# Autodesk Inventor assembly: Ensamble_general
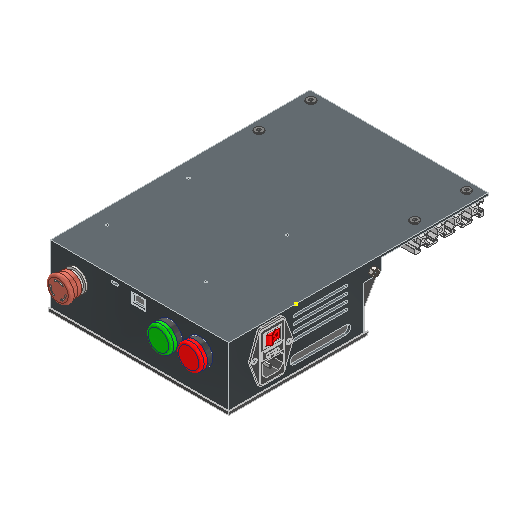
[picture p0: Inventor's stored thumbnail of the model, 512x512]
Saved by Autodesk Inventor 2025 (Build 290162000, 162)
## iProperties
Created: 2026-01-23
Part Number: Ensamble_general
Document SubType Name: Assembly
Designer: HP
Author: HP
## Documents named in this file (24)
- C:\Users\HP\Desktop\TESIS 2\TFC2_20212123_MHinojosa\TFC2-20212123-HW\CAD\Ensamble_general.iam
- C:\Users\HP\Desktop\TESIS 2\TFC2_20212123_MHinojosa\TFC2-20212123-HW\CAD\Chasis\Chasis_CONTROL.ipt
- C:\Users\HP\Desktop\TESIS 2\TFC2_20212123_MHinojosa\TFC2-20212123-HW\CAD\AC_INTERUP\AC_INTERUP.ipt
- C:\Users\HP\Desktop\TESIS 2\TFC2_20212123_MHinojosa\TFC2-20212123-HW\CAD\Banana Socket (Red)\Banana Socket (Red).ipt
- C:\Users\HP\Desktop\TESIS 2\TFC2_20212123_MHinojosa\TFC2-20212123-HW\CAD\Banana Socket (Black)\Banana Socket (Black).ipt
- C:\Users\HP\Desktop\TESIS 2\TFC2_20212123_MHinojosa\TFC2-20212123-HW\CAD\RED LED BULB_F\RED LED BULB_F.ipt
- C:\Users\HP\Desktop\TESIS 2\TFC2_20212123_MHinojosa\TFC2-20212123-HW\CAD\GREEN LED BULB_F\GREEN LED BULB_F.ipt
- C:\Users\HP\Desktop\TESIS 2\TFC2_20212123_MHinojosa\TFC2-20212123-HW\CAD\Profiles\Profiles.ipt
- C:\Users\HP\Desktop\TESIS 2\TFC2_20212123_MHinojosa\TFC2-20212123-HW\CAD\E-Stop\E-Stop.ipt
- C:\Users\HP\Desktop\TESIS 2\TFC2_20212123_MHinojosa\TFC2-20212123-HW\CAD\Tapa_chasis.ipt
- C:\Users\HP\Desktop\TESIS 2\TFC2_20212123_MHinojosa\TFC2-20212123-HW\CAD\BRACKET_MOTOR.ipt
- C:\Users\HP\Desktop\TESIS 2\TFC2_20212123_MHinojosa\TFC2-20212123-HW\CAD\DC Planetary Gear Brush Motor (PZ22GR9120R-084BBH)\DC Planetary Gear Brush Motor (PZ22GR9120R-084BBH).ipt
- C:\Users\HP\Desktop\TESIS 2\TFC2_20212123_MHinojosa\TFC2-20212123-HW\CAD\Slider T-Nut for 2020 - M5\Slider T-Nut for 2020 - M5.ipt
- C:\Users\HP\Desktop\TESIS 2\TFC2_20212123_MHinojosa\TFC2-20212123-HW\CAD\TORNILLO ALLEN CABEZA PLANA M3x0.5x6\TORNILLO ALLEN CABEZA PLANA M5x0.5x6.ipt
- C:\Users\HP\Desktop\TESIS 2\TFC2_20212123_MHinojosa\TFC2-20212123-HW\CAD\BRACKET_SENSOR.ipt
- C:\Users\HP\Desktop\TESIS 2\TFC2_20212123_MHinojosa\TFC2-20212123-HW\CAD\3D_PCB3_2026-01-02\3D_PCB3_2026-01-02.iam
- C:\Users\HP\Desktop\TESIS 2\TFC2_20212123_MHinojosa\TFC2-20212123-HW\CAD\Acople_IMAN_SOLO.ipt
- C:\Users\HP\Desktop\TESIS 2\TFC2_20212123_MHinojosa\TFC2-20212123-HW\CAD\M3x5\M3x5.ipt
- C:\Users\HP\Desktop\TESIS 2\TFC2_20212123_MHinojosa\TFC2-20212123-HW\CAD\M3 nut\M3 nut.ipt
- C:\Users\HP\Desktop\TESIS 2\TFC2_20212123_MHinojosa\TFC2-20212123-HW\CAD\M5x10\M5x10.ipt
- C:\Users\HP\Desktop\TESIS 2\TFC2_20212123_MHinojosa\TFC2-20212123-HW\CAD\M5 Nut\M5 Nut.ipt
- C:\Users\HP\Desktop\TESIS 2\TFC2_20212123_MHinojosa\TFC2-20212123-HW\CAD\M3 x 10 Brass Standoff_\M3 x 10 Brass Standoff_.ipt
- C:\Users\HP\Desktop\TESIS 2\TFC2_20212123_MHinojosa\TFC2-20212123-HW\CAD\3D_PCB10_2026-02-04\3D_PCB10_2026-02-04.ipt
- C:\Users\HP\Desktop\TESIS 2\TFC2_20212123_MHinojosa\TFC2-20212123-HW\CAD\FuenteConmutada24W\FuenteConmutada12V2A\FuenteConmutada12V2A.ipt
## Components (54 placed, 23 different names)
1. Chasis_CONTROL:1 — Coincidencia:1, Coincidencia:2, Coincidencia:3, Coincidencia:9, Coincidencia:10, Coincidencia:11, Coincidencia:12, Nivelación:1, Coincidencia:14, Nivelación:2, Coincidencia:19, Coincidencia:20, Coincidencia:21, Coincidencia:22, Coincidencia:23, Coincidencia:34, Coincidencia:37, Coincidencia:39, Coincidencia:41, Coincidencia:50, Coincidencia:51, Coincidencia:52, Coincidencia:53, Coincidencia:54, Coincidencia:55, Coincidencia:56, Coincidencia:57, Ángulo:1, Ángulo:2, Ángulo:3, Ángulo:4, Ángulo:5, Ángulo:6, Ángulo:7, Ángulo:8, Ángulo:9, Ángulo:10, Coincidencia:124, Coincidencia:127, Coincidencia:129, Coincidencia:134, Coincidencia:135, Ángulo:11, Ángulo:12, Coincidencia:136, Coincidencia:137, Coincidencia:138, Coincidencia:139, Ángulo:13, Ángulo:14, Ángulo:15, Coincidencia:140, Coincidencia:141, Coincidencia:142, Coincidencia:143, Coincidencia:144, Coincidencia:148, Coincidencia:149, Nivelación:13
2. AC_INTERUP:1 — Coincidencia:1, Coincidencia:2, Coincidencia:3
3. RED LED BULB_F:1 — Coincidencia:9, Coincidencia:12, Ángulo:15
4. GREEN LED BULB_F:1 — Coincidencia:10, Coincidencia:11, Ángulo:14
5. Profiles:1 — Nivelación:1, Coincidencia:14, Nivelación:2, Nivelación:5, Coincidencia:28, Nivelación:6, Coincidencia:32, Coincidencia:33, Coincidencia:36, Coincidencia:38, Coincidencia:40, Coincidencia:42, Coincidencia:44, Coincidencia:46, Coincidencia:48, Coincidencia:93, Nivelación:8, Coincidencia:105, Coincidencia:107, Coincidencia:112, Coincidencia:113
6. E-Stop:1 — Coincidencia:19, Coincidencia:20, Ángulo:13
7. Tapa_chasis:1 — Coincidencia:21, Coincidencia:22, Coincidencia:23, Coincidencia:24, Coincidencia:25, Coincidencia:26, Coincidencia:27, Coincidencia:122, Coincidencia:123, Coincidencia:125
8. Banana Socket (Black):2 — Coincidencia:24, Coincidencia:25
9. Banana Socket (Red):2 — Coincidencia:26, Coincidencia:27
10. BRACKET_MOTOR:1 — Nivelación:5, Coincidencia:28, Nivelación:6, Coincidencia:29, Nivelación:7, Coincidencia:43, Coincidencia:45, Coincidencia:47, Coincidencia:49, Coincidencia:58, Coincidencia:59, Coincidencia:60, Coincidencia:61, Coincidencia:62, Coincidencia:63, Coincidencia:64, Coincidencia:65, Nivelación:9
11. DC Planetary Gear Brush Motor (PZ22GR9120R-084BBH):1 — Coincidencia:29, Nivelación:7, Coincidencia:91, Coincidencia:92
12. Slider T-Nut for 2020 - M5:1 — Coincidencia:32, Coincidencia:33, Coincidencia:34, Ángulo:10
13. Slider T-Nut for 2020 - M5:2 — Coincidencia:36, Coincidencia:37, Ángulo:9
14. Slider T-Nut for 2020 - M5:4 — Coincidencia:42, Coincidencia:43, Ángulo:7
15. Slider T-Nut for 2020 - M5:5 — Coincidencia:48, Coincidencia:49, Ángulo:6
16. Slider T-Nut for 2020 - M5:6 — Coincidencia:38, Coincidencia:39, Ángulo:1
17. Slider T-Nut for 2020 - M5:7 — Coincidencia:40, Coincidencia:41, Ángulo:2
18. Slider T-Nut for 2020 - M5:8 — Coincidencia:44, Coincidencia:45, Ángulo:8
19. Slider T-Nut for 2020 - M5:9 — Coincidencia:46, Coincidencia:47, Ángulo:5
20. TORNILLO ALLEN CABEZA PLANA M5x0.5x6:1 — Coincidencia:62, Coincidencia:63
21. TORNILLO ALLEN CABEZA PLANA M5x0.5x6:2 — Coincidencia:56, Coincidencia:57
22. TORNILLO ALLEN CABEZA PLANA M5x0.5x6:3 — Coincidencia:50, Coincidencia:51
23. TORNILLO ALLEN CABEZA PLANA M5x0.5x6:4 — Coincidencia:52, Coincidencia:53
24. TORNILLO ALLEN CABEZA PLANA M5x0.5x6:5 — Coincidencia:64, Coincidencia:65
25. TORNILLO ALLEN CABEZA PLANA M5x0.5x6:7 — Coincidencia:60, Coincidencia:61
26. TORNILLO ALLEN CABEZA PLANA M5x0.5x6:8 — Coincidencia:58, Coincidencia:59
27. TORNILLO ALLEN CABEZA PLANA M5x0.5x6:9 — Coincidencia:54, Coincidencia:55
28. 3D_PCB3_2026-01-02:1 [sub-assembly] — Coincidencia:94, Coincidencia:95, Coincidencia:114, Coincidencia:115, Coincidencia:116, Coincidencia:117
29. Acople_IMAN_SOLO:1 — Coincidencia:91, Coincidencia:92
30. BRACKET_SENSOR:1 — Coincidencia:93, Nivelación:8, Nivelación:9, Coincidencia:94, Coincidencia:95, Coincidencia:96, Coincidencia:97, Coincidencia:98, Coincidencia:99, Coincidencia:100, Coincidencia:101, Coincidencia:102, Coincidencia:103, Coincidencia:118, Coincidencia:120, Coincidencia:126
31. TORNILLO ALLEN CABEZA PLANA M5x0.5x6:10 — Coincidencia:102, Coincidencia:103, Coincidencia:111
32. TORNILLO ALLEN CABEZA PLANA M5x0.5x6:11 — Coincidencia:96, Coincidencia:97, Coincidencia:108
33. TORNILLO ALLEN CABEZA PLANA M5x0.5x6:12 — Coincidencia:98, Coincidencia:99, Coincidencia:110
34. TORNILLO ALLEN CABEZA PLANA M5x0.5x6:14 — Coincidencia:100, Coincidencia:101, Coincidencia:109
35. Slider T-Nut for 2020 - M5:11 — Coincidencia:105, Coincidencia:108, Ángulo:4
36. Slider T-Nut for 2020 - M5:12 — Coincidencia:111, Coincidencia:112, Ángulo:11
37. Slider T-Nut for 2020 - M5:14 — Coincidencia:110, Coincidencia:113, Ángulo:12
38. Slider T-Nut for 2020 - M5:15 — Coincidencia:107, Coincidencia:109, Ángulo:3
39. M3x5:1 — Coincidencia:114, Coincidencia:115, Coincidencia:121, Coincidencia:126
40. M3x5:3 — Coincidencia:116, Coincidencia:117, Coincidencia:119
41. M3 nut:1 — Coincidencia:118, Coincidencia:119
42. M3 nut:3 — Coincidencia:120, Coincidencia:121
43. M5x10:1 — Coincidencia:122, Coincidencia:123, Coincidencia:128
44. M5x10:2 — Coincidencia:124, Coincidencia:125, Coincidencia:130
45. M5 Nut:1 — Coincidencia:127, Coincidencia:128
46. M5 Nut:2 — Coincidencia:129, Coincidencia:130
47. Banana Socket (Black):3 — Coincidencia:137, Coincidencia:138
48. Banana Socket (Red):3 — Coincidencia:136, Coincidencia:139
49. M3 x 10 Brass Standoff_:1 — Nivelación:10, Coincidencia:140, Coincidencia:141, Coincidencia:145
50. M3 x 10 Brass Standoff_:2 — Nivelación:12, Coincidencia:144, Coincidencia:147
51. M3 x 10 Brass Standoff_:3 — Nivelación:11, Nivelación:12, Coincidencia:143, Coincidencia:146
52. M3 x 10 Brass Standoff_:4 — Nivelación:10, Nivelación:11, Coincidencia:142
53. 3D_PCB10_2026-02-04:1 — Coincidencia:145, Coincidencia:146, Coincidencia:147
54. FuenteConmutada12V2A:1 — Coincidencia:148, Coincidencia:149, Nivelación:13
## Relationships (132: Mate 106, Angle 15, Flush 11)
- Coincidencia:1 [Mate]: Chasis_CONTROL:1 ↔ AC_INTERUP:1
- Coincidencia:2 [Mate]: Chasis_CONTROL:1 ↔ AC_INTERUP:1
- Coincidencia:3 [Mate]: Chasis_CONTROL:1 ↔ AC_INTERUP:1
- Coincidencia:9 [Mate]: Chasis_CONTROL:1 ↔ RED LED BULB_F:1
- Coincidencia:10 [Mate]: Chasis_CONTROL:1 ↔ GREEN LED BULB_F:1
- Coincidencia:11 [Mate]: Chasis_CONTROL:1 ↔ GREEN LED BULB_F:1
- Coincidencia:12 [Mate]: Chasis_CONTROL:1 ↔ RED LED BULB_F:1
- Nivelación:1 [Flush] (3 mm): Chasis_CONTROL:1 ↔ Profiles:1
- Coincidencia:14 [Mate]: Chasis_CONTROL:1 ↔ Profiles:1
- Nivelación:2 [Flush] (2 mm): Chasis_CONTROL:1 ↔ Profiles:1
- Coincidencia:19 [Mate]: Chasis_CONTROL:1 ↔ E-Stop:1
- Coincidencia:20 [Mate]: Chasis_CONTROL:1 ↔ E-Stop:1
- Coincidencia:21 [Mate]: Chasis_CONTROL:1 ↔ Tapa_chasis:1
- Coincidencia:22 [Mate]: Chasis_CONTROL:1 ↔ Tapa_chasis:1
- Coincidencia:23 [Mate]: Chasis_CONTROL:1 ↔ Tapa_chasis:1
- Coincidencia:24 [Mate]: Tapa_chasis:1 ↔ Banana Socket (Black):2
- Coincidencia:25 [Mate]: Tapa_chasis:1 ↔ Banana Socket (Black):2
- Coincidencia:26 [Mate]: Tapa_chasis:1 ↔ Banana Socket (Red):2
- Coincidencia:27 [Mate]: Tapa_chasis:1 ↔ Banana Socket (Red):2
- Nivelación:5 [Flush] (20 mm): Profiles:1 ↔ BRACKET_MOTOR:1
- Coincidencia:28 [Mate]: Profiles:1 ↔ BRACKET_MOTOR:1
- Nivelación:6 [Flush] (20 mm): Profiles:1 ↔ BRACKET_MOTOR:1
- Coincidencia:29 [Mate]: BRACKET_MOTOR:1 ↔ DC Planetary Gear Brush Motor (PZ22GR9120R-084BBH):1
- Nivelación:7 [Flush]: BRACKET_MOTOR:1 ↔ DC Planetary Gear Brush Motor (PZ22GR9120R-084BBH):1
- Coincidencia:32 [Mate]: Profiles:1 ↔ Slider T-Nut for 2020 - M5:1
- Coincidencia:33 [Mate]: Profiles:1 ↔ Slider T-Nut for 2020 - M5:1
- Coincidencia:34 [Mate]: Chasis_CONTROL:1 ↔ Slider T-Nut for 2020 - M5:1
- Coincidencia:36 [Mate]: Profiles:1 ↔ Slider T-Nut for 2020 - M5:2
- Coincidencia:37 [Mate]: Chasis_CONTROL:1 ↔ Slider T-Nut for 2020 - M5:2
- Coincidencia:38 [Mate]: Profiles:1 ↔ Slider T-Nut for 2020 - M5:6
- Coincidencia:39 [Mate]: Chasis_CONTROL:1 ↔ Slider T-Nut for 2020 - M5:6
- Coincidencia:40 [Mate]: Profiles:1 ↔ Slider T-Nut for 2020 - M5:7
- Coincidencia:41 [Mate]: Chasis_CONTROL:1 ↔ Slider T-Nut for 2020 - M5:7
- Coincidencia:42 [Mate]: Profiles:1 ↔ Slider T-Nut for 2020 - M5:4
- Coincidencia:43 [Mate]: BRACKET_MOTOR:1 ↔ Slider T-Nut for 2020 - M5:4
- Coincidencia:44 [Mate]: Profiles:1 ↔ Slider T-Nut for 2020 - M5:8
- Coincidencia:45 [Mate]: BRACKET_MOTOR:1 ↔ Slider T-Nut for 2020 - M5:8
- Coincidencia:46 [Mate]: Profiles:1 ↔ Slider T-Nut for 2020 - M5:9
- Coincidencia:47 [Mate]: BRACKET_MOTOR:1 ↔ Slider T-Nut for 2020 - M5:9
- Coincidencia:48 [Mate]: Profiles:1 ↔ Slider T-Nut for 2020 - M5:5
- Coincidencia:49 [Mate]: BRACKET_MOTOR:1 ↔ Slider T-Nut for 2020 - M5:5
- Coincidencia:50 [Mate] (1 mm): Chasis_CONTROL:1 ↔ TORNILLO ALLEN CABEZA PLANA M5x0.5x6:3
- Coincidencia:51 [Mate]: Chasis_CONTROL:1 ↔ TORNILLO ALLEN CABEZA PLANA M5x0.5x6:3
- Coincidencia:52 [Mate]: Chasis_CONTROL:1 ↔ TORNILLO ALLEN CABEZA PLANA M5x0.5x6:4
- Coincidencia:53 [Mate] (1 mm): Chasis_CONTROL:1 ↔ TORNILLO ALLEN CABEZA PLANA M5x0.5x6:4
- Coincidencia:54 [Mate]: Chasis_CONTROL:1 ↔ TORNILLO ALLEN CABEZA PLANA M5x0.5x6:9
- Coincidencia:55 [Mate] (1 mm): Chasis_CONTROL:1 ↔ TORNILLO ALLEN CABEZA PLANA M5x0.5x6:9
- Coincidencia:56 [Mate]: Chasis_CONTROL:1 ↔ TORNILLO ALLEN CABEZA PLANA M5x0.5x6:2
- Coincidencia:57 [Mate] (1 mm): Chasis_CONTROL:1 ↔ TORNILLO ALLEN CABEZA PLANA M5x0.5x6:2
- Coincidencia:58 [Mate]: BRACKET_MOTOR:1 ↔ TORNILLO ALLEN CABEZA PLANA M5x0.5x6:8
- Coincidencia:59 [Mate] (1 mm): BRACKET_MOTOR:1 ↔ TORNILLO ALLEN CABEZA PLANA M5x0.5x6:8
- Coincidencia:60 [Mate]: BRACKET_MOTOR:1 ↔ TORNILLO ALLEN CABEZA PLANA M5x0.5x6:7
- Coincidencia:61 [Mate] (1 mm): BRACKET_MOTOR:1 ↔ TORNILLO ALLEN CABEZA PLANA M5x0.5x6:7
- Coincidencia:62 [Mate]: BRACKET_MOTOR:1 ↔ TORNILLO ALLEN CABEZA PLANA M5x0.5x6:1
- Coincidencia:63 [Mate] (1 mm): BRACKET_MOTOR:1 ↔ TORNILLO ALLEN CABEZA PLANA M5x0.5x6:1
- Coincidencia:64 [Mate]: BRACKET_MOTOR:1 ↔ TORNILLO ALLEN CABEZA PLANA M5x0.5x6:5
- Coincidencia:65 [Mate] (1 mm): BRACKET_MOTOR:1 ↔ TORNILLO ALLEN CABEZA PLANA M5x0.5x6:5
- Coincidencia:91 [Mate]: DC Planetary Gear Brush Motor (PZ22GR9120R-084BBH):1 ↔ Acople_IMAN_SOLO:1
- Coincidencia:92 [Mate]: DC Planetary Gear Brush Motor (PZ22GR9120R-084BBH):1 ↔ Acople_IMAN_SOLO:1
- Coincidencia:93 [Mate]: Profiles:1 ↔ BRACKET_SENSOR:1
- Nivelación:8 [Flush] (76.151 mm): Profiles:1 ↔ BRACKET_SENSOR:1
- Nivelación:9 [Flush]: BRACKET_MOTOR:1 ↔ BRACKET_SENSOR:1
- Coincidencia:94 [Mate]: 3D_PCB3_2026-01-02:1 ↔ BRACKET_SENSOR:1
- Coincidencia:95 [Mate]: 3D_PCB3_2026-01-02:1 ↔ BRACKET_SENSOR:1
- Coincidencia:96 [Mate]: BRACKET_SENSOR:1 ↔ TORNILLO ALLEN CABEZA PLANA M5x0.5x6:11
- Coincidencia:97 [Mate] (2 mm): BRACKET_SENSOR:1 ↔ TORNILLO ALLEN CABEZA PLANA M5x0.5x6:11
- Coincidencia:98 [Mate] (2 mm): BRACKET_SENSOR:1 ↔ TORNILLO ALLEN CABEZA PLANA M5x0.5x6:12
- Coincidencia:99 [Mate]: BRACKET_SENSOR:1 ↔ TORNILLO ALLEN CABEZA PLANA M5x0.5x6:12
- Coincidencia:100 [Mate]: BRACKET_SENSOR:1 ↔ TORNILLO ALLEN CABEZA PLANA M5x0.5x6:14
- Coincidencia:101 [Mate] (2 mm): BRACKET_SENSOR:1 ↔ TORNILLO ALLEN CABEZA PLANA M5x0.5x6:14
- Coincidencia:102 [Mate]: BRACKET_SENSOR:1 ↔ TORNILLO ALLEN CABEZA PLANA M5x0.5x6:10
- Coincidencia:103 [Mate] (2 mm): BRACKET_SENSOR:1 ↔ TORNILLO ALLEN CABEZA PLANA M5x0.5x6:10
- Coincidencia:105 [Mate]: Profiles:1 ↔ Slider T-Nut for 2020 - M5:11
- Coincidencia:107 [Mate]: Profiles:1 ↔ Slider T-Nut for 2020 - M5:15
- Coincidencia:108 [Mate]: TORNILLO ALLEN CABEZA PLANA M5x0.5x6:11 ↔ Slider T-Nut for 2020 - M5:11
- Coincidencia:109 [Mate]: TORNILLO ALLEN CABEZA PLANA M5x0.5x6:14 ↔ Slider T-Nut for 2020 - M5:15
- Coincidencia:110 [Mate]: TORNILLO ALLEN CABEZA PLANA M5x0.5x6:12 ↔ Slider T-Nut for 2020 - M5:14
- Coincidencia:111 [Mate]: TORNILLO ALLEN CABEZA PLANA M5x0.5x6:10 ↔ Slider T-Nut for 2020 - M5:12
- Coincidencia:112 [Mate]: Profiles:1 ↔ Slider T-Nut for 2020 - M5:12
- Coincidencia:113 [Mate]: Profiles:1 ↔ Slider T-Nut for 2020 - M5:14
- Ángulo:1 [Angle] (0 deg): Chasis_CONTROL:1 ↔ Slider T-Nut for 2020 - M5:6
- Ángulo:2 [Angle] (0 deg): Chasis_CONTROL:1 ↔ Slider T-Nut for 2020 - M5:7
- Ángulo:3 [Angle] (0 deg): Chasis_CONTROL:1 ↔ Slider T-Nut for 2020 - M5:15
- Ángulo:4 [Angle] (0 deg): Chasis_CONTROL:1 ↔ Slider T-Nut for 2020 - M5:11
- Ángulo:5 [Angle] (0 deg): Chasis_CONTROL:1 ↔ Slider T-Nut for 2020 - M5:9
- Ángulo:6 [Angle] (0 deg): Chasis_CONTROL:1 ↔ Slider T-Nut for 2020 - M5:5
- Ángulo:7 [Angle] (0 deg): Chasis_CONTROL:1 ↔ Slider T-Nut for 2020 - M5:4
- Ángulo:8 [Angle] (0 deg): Chasis_CONTROL:1 ↔ Slider T-Nut for 2020 - M5:8
- Ángulo:9 [Angle] (0 deg): Chasis_CONTROL:1 ↔ Slider T-Nut for 2020 - M5:2
- Ángulo:10 [Angle] (0 deg): Chasis_CONTROL:1 ↔ Slider T-Nut for 2020 - M5:1
- Coincidencia:114 [Mate]: 3D_PCB3_2026-01-02:1 ↔ M3x5:1
- Coincidencia:115 [Mate]: 3D_PCB3_2026-01-02:1 ↔ M3x5:1
- Coincidencia:116 [Mate]: 3D_PCB3_2026-01-02:1 ↔ M3x5:3
- Coincidencia:117 [Mate]: 3D_PCB3_2026-01-02:1 ↔ M3x5:3
- Coincidencia:118 [Mate]: BRACKET_SENSOR:1 ↔ M3 nut:1
- Coincidencia:119 [Mate]: M3x5:3 ↔ M3 nut:1
- Coincidencia:120 [Mate]: BRACKET_SENSOR:1 ↔ M3 nut:3
- Coincidencia:121 [Mate]: M3x5:1 ↔ M3 nut:3
- Coincidencia:122 [Mate]: Tapa_chasis:1 ↔ M5x10:1
- Coincidencia:123 [Mate]: Tapa_chasis:1 ↔ M5x10:1
- Coincidencia:124 [Mate]: Chasis_CONTROL:1 ↔ M5x10:2
- Coincidencia:125 [Mate]: Tapa_chasis:1 ↔ M5x10:2
- Coincidencia:126 [Mate]: BRACKET_SENSOR:1 ↔ M3x5:1
- Coincidencia:127 [Mate]: Chasis_CONTROL:1 ↔ M5 Nut:1
- Coincidencia:128 [Mate]: M5x10:1 ↔ M5 Nut:1
- Coincidencia:129 [Mate]: Chasis_CONTROL:1 ↔ M5 Nut:2
- Coincidencia:130 [Mate]: M5x10:2 ↔ M5 Nut:2
- Coincidencia:134 [Mate]: Chasis_CONTROL:1
- Coincidencia:135 [Mate]: Chasis_CONTROL:1
- Ángulo:11 [Angle] (0 deg): Chasis_CONTROL:1 ↔ Slider T-Nut for 2020 - M5:12
- Ángulo:12 [Angle] (0 deg): Chasis_CONTROL:1 ↔ Slider T-Nut for 2020 - M5:14
- Coincidencia:136 [Mate]: Chasis_CONTROL:1 ↔ Banana Socket (Red):3
- Coincidencia:137 [Mate]: Chasis_CONTROL:1 ↔ Banana Socket (Black):3
- Coincidencia:138 [Mate]: Chasis_CONTROL:1 ↔ Banana Socket (Black):3
- Coincidencia:139 [Mate]: Chasis_CONTROL:1 ↔ Banana Socket (Red):3
- Ángulo:13 [Angle] (0 deg): Chasis_CONTROL:1 ↔ E-Stop:1
- Ángulo:14 [Angle] (0 deg): Chasis_CONTROL:1 ↔ GREEN LED BULB_F:1
- Ángulo:15 [Angle] (0 deg): Chasis_CONTROL:1 ↔ RED LED BULB_F:1
- Nivelación:10 [Flush]: M3 x 10 Brass Standoff_:1 ↔ M3 x 10 Brass Standoff_:4
- Nivelación:11 [Flush]: M3 x 10 Brass Standoff_:3 ↔ M3 x 10 Brass Standoff_:4
- Nivelación:12 [Flush]: M3 x 10 Brass Standoff_:2 ↔ M3 x 10 Brass Standoff_:3
- Coincidencia:140 [Mate]: Chasis_CONTROL:1 ↔ M3 x 10 Brass Standoff_:1
- Coincidencia:141 [Mate]: Chasis_CONTROL:1 ↔ M3 x 10 Brass Standoff_:1
- Coincidencia:142 [Mate]: Chasis_CONTROL:1 ↔ M3 x 10 Brass Standoff_:4
- Coincidencia:143 [Mate]: Chasis_CONTROL:1 ↔ M3 x 10 Brass Standoff_:3
- Coincidencia:144 [Mate]: Chasis_CONTROL:1 ↔ M3 x 10 Brass Standoff_:2
- Coincidencia:145 [Mate]: M3 x 10 Brass Standoff_:1 ↔ 3D_PCB10_2026-02-04:1
- Coincidencia:146 [Mate]: M3 x 10 Brass Standoff_:3 ↔ 3D_PCB10_2026-02-04:1
- Coincidencia:147 [Mate]: M3 x 10 Brass Standoff_:2 ↔ 3D_PCB10_2026-02-04:1
- Coincidencia:148 [Mate]: Chasis_CONTROL:1 ↔ FuenteConmutada12V2A:1
- Coincidencia:149 [Mate]: Chasis_CONTROL:1 ↔ FuenteConmutada12V2A:1
- Nivelación:13 [Flush] (-22 mm): Chasis_CONTROL:1 ↔ FuenteConmutada12V2A:1
